# Autodesk Inventor assembly: Baugruppe1
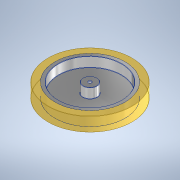
[picture p0: Inventor's stored thumbnail of the model, 180x180]
Saved by Autodesk Inventor 2022 (Build 260153000, 153)
## iProperties
Created: 2022-11-16
Part Number: Baugruppe1
Document SubType Name: Assembly
Designer: Friedrich Walmrath
Author: Friedrich Walmrath
## Documents named in this file (9)
- E:\InventorProjekte\karten schießer\v2\simtest\Baugruppe1.iam
- E:\InventorProjekte\karten schießer\v2\simtest\felge.ipt
- E:\InventorProjekte\karten schießer\v2\simtest\reifen.ipt
- E:\InventorProjekte\karten schießer\v2\simtest\Baugruppe1\AIP\FEA\e5l65niao.fins
- E:\InventorProjekte\karten schießer\v2\simtest\Baugruppe1\AIP\FEA\e5l65niao.fsat
- E:\InventorProjekte\karten schießer\v2\simtest\Baugruppe1\AIP\FEA\e5l65niao.ftes
- E:\InventorProjekte\karten schießer\v2\simtest\Baugruppe1\AIP\FEA\e5l65niao.fwiz
- E:\InventorProjekte\karten schießer\v2\simtest\Baugruppe1\AIP\FEA\e5l65nibk.fmsh
- E:\InventorProjekte\karten schießer\v2\simtest\Baugruppe1\AIP\FEA\e5l65nibl.fres
## Components (2 placed, 2 different names)
1. felge:1
2. reifen:1
## Named parameters: sa_0 = 2792.53, sa_1 = 0
note: some values were not read from the file. Shown as the stored number, unit unknown: "sa_0", "sa_1".
